# Autodesk Inventor assembly: Assembly1
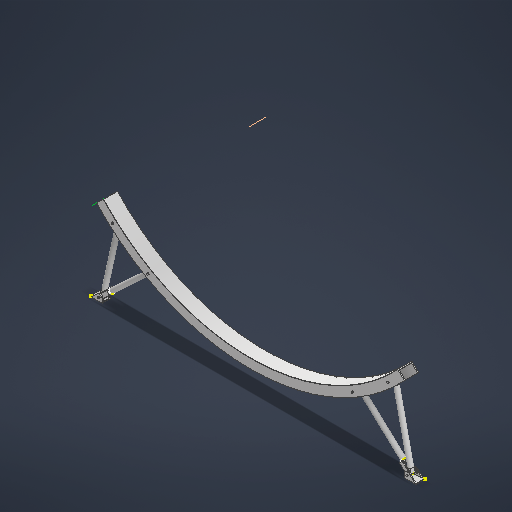
[picture p0: Inventor's stored thumbnail of the model, 512x512]
Saved by Autodesk Inventor 2026.1 (Build 301233020, 233B)
## iProperties
Created: 2025-11-07
Part Number: Assembly1
Document SubType Name: Assembly
Designer: Study
Author: Study
## Documents named in this file (8)
- C:\Users\Study\Desktop\Alec's Games\folder\3D Files\Assembly1.iam
- C:\Users\Study\Desktop\Alec's Games\folder\3D Files\Sled.ipt
- C:\Users\Study\Desktop\Alec's Games\folder\3D Files\Leg.ipt
- C:\Users\Study\Desktop\Alec's Games\folder\3D Files\LegSecondary.ipt
- C:\Users\Study\Desktop\Alec's Games\folder\3D Files\BoltM10_150.ipt
- C:\Users\Study\Desktop\Alec's Games\folder\3D Files\BoltM10_90.ipt
- C:\Users\Study\Desktop\Alec's Games\folder\3D Files\NutM10.ipt
- C:\Users\Study\Desktop\Alec's Games\folder\3D Files\Foot.ipt
## Components (19 placed, 7 different names)
1. Sled:1 — Rotational:1, Rotational:2, Rotational:3, Rotational:4, Rotational:7, Rotational:8, Rotational:9, Rotational:10
2. Leg:1 — Rotational:1, Rotational:5
3. Leg:2 — Rotational:2, Rotational:6
4. LegSecondary:1 — Rotational:3, Rotational:5, Rotational:12
5. LegSecondary:2 — Rotational:4, Rotational:6, Rotational:14
6. BoltM10_150:1 — Rotational:7, Rotational:11
7. BoltM10_150:2 — Rotational:8, Rigid:3
8. BoltM10_150:3 — Rotational:9, Rigid:2
9. BoltM10_150:4 — Rotational:10, Rigid:1
10. BoltM10_90:1 — Rotational:15, Rigid:5
11. BoltM10_90:2 — Rotational:13, Rigid:4
12. NutM10:1 — Rigid:5
13. NutM10:2 — Rigid:4
14. NutM10:3 — Rigid:1
15. NutM10:4 — Rigid:2
16. NutM10:5 — Rigid:3
17. NutM10:6 — Rotational:11
18. Foot:1 — Rotational:14, Rotational:15
19. Foot:2 — Rotational:12, Rotational:13
## Relationships (20: RevoluteJoint 15, WeldJoint 5)
- Rotational:1 [RevoluteJoint]: Sled:1 ↔ Leg:1
- Rotational:2 [RevoluteJoint]: Sled:1 ↔ Leg:2
- Rotational:3 [RevoluteJoint]: Sled:1 ↔ LegSecondary:1
- Rotational:4 [RevoluteJoint]: Sled:1 ↔ LegSecondary:2
- Rotational:5 [RevoluteJoint]: Leg:1 ↔ LegSecondary:1
- Rotational:6 [RevoluteJoint]: Leg:2 ↔ LegSecondary:2
- Rotational:7 [RevoluteJoint]: Sled:1 ↔ BoltM10_150:1
- Rotational:8 [RevoluteJoint]: Sled:1 ↔ BoltM10_150:2
- Rotational:9 [RevoluteJoint]: Sled:1 ↔ BoltM10_150:3
- Rotational:10 [RevoluteJoint]: Sled:1 ↔ BoltM10_150:4
- Rigid:1 [WeldJoint]: BoltM10_150:4 ↔ NutM10:3
- Rigid:2 [WeldJoint]: BoltM10_150:3 ↔ NutM10:4
- Rigid:3 [WeldJoint]: BoltM10_150:2 ↔ NutM10:5
- Rotational:11 [RevoluteJoint]: BoltM10_150:1 ↔ NutM10:6
- Rotational:12 [RevoluteJoint]: LegSecondary:1 ↔ Foot:2
- Rotational:13 [RevoluteJoint]: BoltM10_90:2 ↔ Foot:2
- Rigid:4 [WeldJoint]: BoltM10_90:2 ↔ NutM10:2
- Rotational:14 [RevoluteJoint]: LegSecondary:2 ↔ Foot:1
- Rotational:15 [RevoluteJoint]: BoltM10_90:1 ↔ Foot:1
- Rigid:5 [WeldJoint]: BoltM10_90:1 ↔ NutM10:1
